# Autodesk Inventor assembly: belt_curve
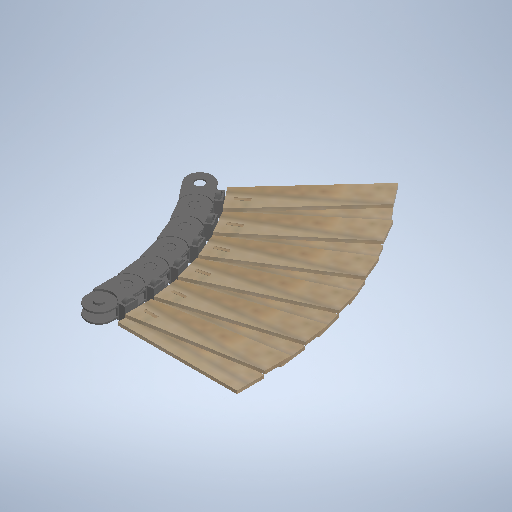
[picture p0: Inventor's stored thumbnail of the model, 512x512]
Saved by Autodesk Inventor 2026.1 (Build 301233020, 233B)
## iProperties
Created: 2025-09-28
Part Number: belt_curve
Document SubType Name: Assembly
Designer: hibik
Author: hibik
## Documents named in this file (3)
- C:\Users\hibik\Documents\Robomech\conveyer\belt\belt_curve.iam
- C:\Users\hibik\Documents\Robomech\conveyer\belt\belt.ipt
- C:\Users\hibik\Documents\Robomech\conveyer\belt\dish.iam
## Components (12 placed, 2 different names)
1. belt:1 — 挿入:1, 角度:1, メイト:1, メイト:7, メイト:13
2. belt:2 — 挿入:1, 挿入:2, 角度:1, 角度:2, メイト:2, メイト:8, メイト:14
3. belt:3 — 挿入:2, 挿入:3, 角度:2, 角度:3, メイト:3, メイト:9, メイト:15
4. belt:4 — 挿入:3, 挿入:4, 角度:3, 角度:4, メイト:4, メイト:10, メイト:16
5. belt:5 — 挿入:4, 挿入:5, 角度:4, 角度:5, メイト:5, メイト:11, メイト:17
6. belt:6 — 挿入:5, 角度:5, メイト:6, メイト:12, メイト:18
7. dish:1 [sub-assembly] — メイト:1, メイト:7, メイト:13
8. dish:2 [sub-assembly] — メイト:3, メイト:9, メイト:15
9. dish:3 [sub-assembly] — メイト:2, メイト:8, メイト:14
10. dish:4 [sub-assembly] — メイト:6, メイト:12, メイト:18
11. dish:5 [sub-assembly] — メイト:5, メイト:11, メイト:17
12. dish:6 [sub-assembly] — メイト:4, メイト:10, メイト:16
## Relationships (28: Mate 18, Insert 5, Angle 5)
- 挿入:1 [Insert] (0.6 mm): belt:1 ↔ belt:2
- 挿入:2 [Insert] (0.6 mm): belt:2 ↔ belt:3
- 挿入:3 [Insert] (0.6 mm): belt:3 ↔ belt:4
- 挿入:4 [Insert] (0.6 mm): belt:4 ↔ belt:5
- 挿入:5 [Insert] (0.6 mm): belt:5 ↔ belt:6
- 角度:1 [Angle] (-7.5 deg): belt:1 ↔ belt:2
- 角度:2 [Angle] (-7.5 deg): belt:2 ↔ belt:3
- 角度:3 [Angle] (-7.5 deg): belt:3 ↔ belt:4
- 角度:4 [Angle] (-7.5 deg): belt:4 ↔ belt:5
- 角度:5 [Angle] (7.5 deg): belt:5 ↔ belt:6
- メイト:1 [Mate]: belt:1 ↔ dish:1
- メイト:2 [Mate]: belt:2 ↔ dish:3
- メイト:3 [Mate]: belt:3 ↔ dish:2
- メイト:4 [Mate]: belt:4 ↔ dish:6
- メイト:5 [Mate]: belt:5 ↔ dish:5
- メイト:6 [Mate]: belt:6 ↔ dish:4
- メイト:7 [Mate]: belt:1 ↔ dish:1
- メイト:8 [Mate]: belt:2 ↔ dish:3
- メイト:9 [Mate]: belt:3 ↔ dish:2
- メイト:10 [Mate]: belt:4 ↔ dish:6
- メイト:11 [Mate]: belt:5 ↔ dish:5
- メイト:12 [Mate]: belt:6 ↔ dish:4
- メイト:13 [Mate]: belt:1 ↔ dish:1
- メイト:14 [Mate]: belt:2 ↔ dish:3
- メイト:15 [Mate]: belt:3 ↔ dish:2
- メイト:16 [Mate]: belt:4 ↔ dish:6
- メイト:17 [Mate]: belt:5 ↔ dish:5
- メイト:18 [Mate]: belt:6 ↔ dish:4
